# Autodesk Inventor assembly: assembly
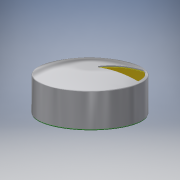
[picture p0: Inventor's stored thumbnail of the model, 180x180]
Saved by Autodesk Inventor 2019 (Build 230136000, 136)
## iProperties
Created: 2019-04-09
Part Number: assembly
Document SubType Name: Assembly
Designer: jmc
Author: jmc
## Documents named in this file (7)
- D:\Inventor\Projects\CatFeeder\Case\version7\assembly.iam
- D:\Inventor\Projects\CatFeeder\Case\version7\inner_case.ipt
- D:\Inventor\Projects\CatFeeder\Case\version7\cap.ipt
- D:\Inventor\Projects\CatFeeder\Case\version7\base.ipt
- D:\Inventor\Projects\CatFeeder\Case\version7\motor_support.ipt
- D:\Inventor\Projects\CatFeeder\Case\version7\motordriver_footprint.ipt
- D:\Inventor\Projects\CatFeeder\Case\version7\esp8266_footprint.ipt
## Components (6 placed, 6 different names)
1. inner_case:1 — Rotational:1, Rigid:1, Rigid:2, Rigid:3, Rigid:4
2. cap:1 — Rotational:1
3. base:1 — Rigid:1
4. motor_support:1 — Rigid:2
5. motordriver_footprint:1 — Rigid:4
6. esp8266_footprint:1 — Rigid:3
## Relationships (5: WeldJoint 4, RevoluteJoint 1)
- Rotational:1 [RevoluteJoint] (2 mm): inner_case:1 ↔ cap:1
- Rigid:1 [WeldJoint]: inner_case:1 ↔ base:1
- Rigid:2 [WeldJoint]: inner_case:1 ↔ motor_support:1
- Rigid:3 [WeldJoint]: inner_case:1 ↔ esp8266_footprint:1
- Rigid:4 [WeldJoint]: inner_case:1 ↔ motordriver_footprint:1
